# Autodesk Inventor assembly: 276-2185
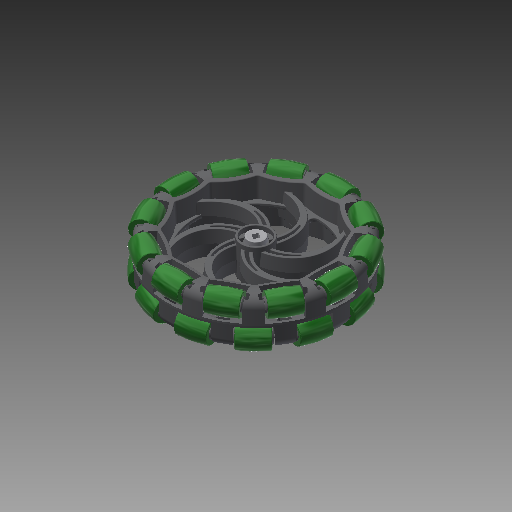
[picture p0: Inventor's stored thumbnail of the model, 512x512]
Saved by Autodesk Inventor 2019 (Build 230136000, 136)
## iProperties
Category: Motion
Company: Autodesk Inc.
Created: 2012-03-14
Part Number: 276-2185
Document SubType Name: Assembly
Designer: Autodesk Inc.
Catalog Web Link: http://www.vexrobotics.com/276-2185.html#
Vendor: VEX
Author: Autodesk Inc.
## Documents named in this file (4)
- F:\VEX Inventor Library\VEX Parts Library 2016\Imperial\Motion\4 inch Omni Directional Wheel.iam
- F:\VEX Inventor Library\VEX Parts Library 2016\Imperial\Motion\Components\LARGE-OMNI-HUB-INSERT.ipt
- F:\VEX Inventor Library\VEX Parts Library 2016\Imperial\Motion\Components\LARGE-OMNI-HUB.ipt
- F:\VEX Inventor Library\VEX Parts Library 2016\Imperial\Motion\Components\Omni Roller.iam
## Components (3 placed, 3 different names)
1. LARGE-OMNI-HUB:1 — Mate:1, Mate:2
2. LARGE-OMNI-HUB-INSERT:1
3. Omni Roller:1 [sub-assembly] — Mate:1, Mate:2
## Relationships (2: Mate 2)
- Mate:1: LARGE-OMNI-HUB:1 ↔ Omni Roller:1
- Mate:2: LARGE-OMNI-HUB:1 ↔ Omni Roller:1
